# Autodesk Inventor assembly: 조립품2
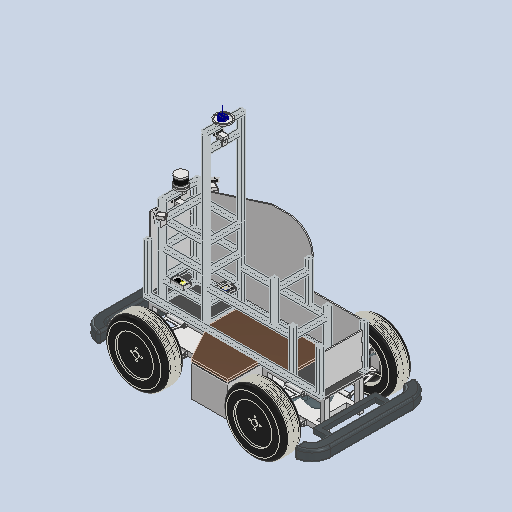
[picture p0: Inventor's stored thumbnail of the model, 512x512]
Saved by Autodesk Inventor 2025.2 (Build 292293000, 293)
## iProperties
Created: 2025-01-26
Part Number: 조립품2
Document SubType Name: Assembly
Designer: jbhma
Author: jbhma
## Documents named in this file (38)
- C:\Users\jbhma\OneDrive\Desktop\2025_ACCA\2024 ERP42\25_Car\Car - 복사본.iam
- C:\Users\jbhma\OneDrive\Desktop\2025_ACCA\2024 ERP42\body.ipt
- C:\Users\jbhma\OneDrive\Desktop\2025_ACCA\2024 ERP42\body_braket.ipt
- C:\Users\jbhma\OneDrive\Desktop\2025_ACCA\2024 ERP42\프로파일\40.5.ipt
- C:\Users\jbhma\OneDrive\Desktop\2025_ACCA\2024 ERP42\프로파일\71.ipt
- C:\Users\jbhma\OneDrive\Desktop\2025_ACCA\2024 ERP42\프로파일\34.ipt
- C:\Users\jbhma\OneDrive\Desktop\2025_ACCA\2024 ERP42\프로파일\26.ipt
- C:\Users\jbhma\OneDrive\Desktop\2025_ACCA\2024 ERP42\프로파일\79.ipt
- C:\Users\jbhma\OneDrive\Desktop\2025_ACCA\2024 ERP42\프로파일\39.ipt
- C:\Users\jbhma\OneDrive\Desktop\2025_ACCA\2024 ERP42\bumper.ipt
- C:\Users\jbhma\OneDrive\Desktop\2025_ACCA\2024 ERP42\link.ipt
- C:\Users\jbhma\OneDrive\Desktop\2025_ACCA\2024 ERP42\wheel_bolt.ipt
- C:\Users\jbhma\OneDrive\Desktop\2025_ACCA\2024 ERP42\wheel_braket_13.ipt
- C:\Users\jbhma\OneDrive\Desktop\2025_ACCA\2024 ERP42\wheel_braket_24.ipt
- C:\Users\jbhma\OneDrive\Desktop\2025_ACCA\2024 ERP42\wheel.ipt
- C:\Users\jbhma\OneDrive\Desktop\2025_ACCA\2024 ERP42\base_link.ipt
- base_link.ipt
- C:\Users\jbhma\OneDrive\Desktop\2025_ACCA\2024 ERP42\프로파일\50.ipt
- C:\Users\jbhma\OneDrive\Desktop\2025_ACCA\2024 ERP42\camera_case_front.ipt
- C:\Users\jbhma\OneDrive\Desktop\2025_ACCA\2024 ERP42\camera_case_left.ipt
- C:\Users\jbhma\OneDrive\Desktop\2025_ACCA\2024 ERP42\camera_case_right.ipt
- C:\Users\jbhma\OneDrive\Desktop\2025_ACCA\2024 ERP42\camera.ipt
- C:\Users\jbhma\OneDrive\Desktop\2025_ACCA\2024 ERP42\lidar_case.ipt
- C:\Users\jbhma\OneDrive\Desktop\2025_ACCA\2024 ERP42\imu_case_new.ipt
- C:\Users\jbhma\OneDrive\Desktop\2025_ACCA\2024 ERP42\gps_case.ipt
- C:\Users\jbhma\OneDrive\Desktop\2025_ACCA\2024 ERP42\UBLOX_ANN-MB-00_GNSS_ANTENNA.ipt
- C:\Users\jbhma\OneDrive\Desktop\2025_ACCA\2024 ERP42\lidar.ipt
- C:\Users\jbhma\OneDrive\Desktop\2025_ACCA\2024 ERP42\MTi 600-series STEP files\MTi-600 DEV assembly.iam
- C:\Users\jbhma\OneDrive\Desktop\2025_ACCA\2024 ERP42\MTi 600-series STEP files\MTi 1-s DK GNSS.iam
- C:\Users\jbhma\OneDrive\Desktop\2025_ACCA\2024 ERP42\gps_case_2.ipt
- C:\Users\jbhma\OneDrive\Desktop\2025_ACCA\2024 ERP42\gps_black.ipt
- C:\Users\jbhma\OneDrive\Desktop\2025_ACCA\2024 ERP42\cover.ipt
- C:\Users\jbhma\OneDrive\Desktop\2025_ACCA\2024 ERP42\고무커버.ipt
- C:\Users\jbhma\OneDrive\Desktop\2025_ACCA\2024 ERP42\프로파일\153.ipt
- C:\Users\jbhma\OneDrive\Desktop\2025_ACCA\2024 ERP42\side_cowl.ipt
- C:\Users\jbhma\OneDrive\Desktop\2025_ACCA\2024 ERP42\back_cowl.ipt
- C:\Users\jbhma\OneDrive\Desktop\2025_ACCA\2024 ERP42\fornt_cowl.ipt
- C:\Users\jbhma\OneDrive\Desktop\2025_ACCA\2024 ERP42\프로파일\34.5.ipt
## Components (101 placed, 36 different names)
1. body:1 — 메이트:113, 메이트:114, 메이트:115, 메이트:116, 메이트:117, 메이트:118, 메이트:119, 메이트:120, 메이트:124, 메이트:125, 메이트:126, 메이트:127, 메이트:128, 메이트:131, 메이트:137, 메이트:139, 메이트:159, 메이트:162, 메이트:191, 메이트:192, 메이트:193, 메이트:194, 메이트:195, 메이트:196, 메이트:197, 메이트:198, 메이트:199, 메이트:200, 메이트:201, 메이트:202, 메이트:203, 메이트:204, 메이트:205, 메이트:206, 메이트:303, 메이트:348, 메이트:349
2. body_braket:9 — 메이트:113, 메이트:114, 메이트:212
3. body_braket:10 — 메이트:115, 메이트:116, 메이트:211
4. body_braket:11 — 메이트:117, 메이트:118, 메이트:213
5. body_braket:12 — 메이트:119, 메이트:120, 메이트:214
6. body_braket:13 — 메이트:191, 메이트:195, 메이트:199, 메이트:215
7. body_braket:14 — 메이트:193, 메이트:197, 메이트:202, 메이트:217
8. body_braket:15 — 메이트:194, 메이트:198, 메이트:201, 메이트:218
9. body_braket:16 — 메이트:192, 메이트:196, 메이트:200, 메이트:216
10. bumper:1 — 메이트:203, 메이트:204
11. bumper:2 — 메이트:205, 메이트:206
12. 40.5:12 — 메이트:126, 메이트:127, 메이트:130, 메이트:257
13. 40.5:13 — 메이트:124, 메이트:125, 메이트:129
14. 71:1 — 메이트:128, 메이트:129, 메이트:132, 메이트:133, 메이트:138
15. 71:2 — 메이트:130, 메이트:131, 메이트:134, 메이트:135, 메이트:136, 메이트:256
16. 34:1 — 메이트:134, 메이트:135, 메이트:189
17. 34:2 — 메이트:132, 메이트:133, 메이트:190
18. 40.5:15 — 메이트:136, 메이트:137, 메이트:143, 메이트:144, 메이트:145, 메이트:326
19. 40.5:16 — 메이트:138, 메이트:139, 메이트:140, 메이트:141, 메이트:142, 메이트:155, 메이트:287, 메이트:288, 메이트:324, 메이트:332
20. 26:1 — 메이트:140, 메이트:141, 메이트:142, 메이트:149, 메이트:150, 메이트:156, 메이트:175, 메이트:176, 메이트:178
21. 26:2 — 메이트:143, 메이트:144, 메이트:145, 메이트:151, 메이트:152, 메이트:157, 메이트:158, 메이트:177
22. 79:1 — 메이트:151, 메이트:152, 메이트:261
23. 79:2 — 메이트:149, 메이트:150, 메이트:153, 메이트:154, 메이트:262, 각도:3
24. 34:3 — 메이트:153, 메이트:154, 메이트:259
25. 34:4 — 메이트:155, 메이트:156, 메이트:160, 메이트:174
26. 34:5 — 메이트:157, 메이트:158, 메이트:161
27. 40.5:17 — 메이트:161, 메이트:162, 메이트:163, 메이트:164, 메이트:282, 메이트:304
28. 40.5:18 — 메이트:159, 메이트:160, 메이트:165, 메이트:166, 메이트:283, 메이트:330
29. 39:1 — 메이트:163, 메이트:164, 메이트:183, 메이트:187
30. 39:2 — 메이트:165, 메이트:166, 메이트:173, 메이트:185, 메이트:252, 메이트:253, 메이트:266, 메이트:347
31. 26:4 — 메이트:173, 메이트:174
32. 26:5 — 메이트:175, 메이트:176
33. 26:6 — 메이트:177, 메이트:178, 메이트:182, 메이트:184
34. 26:8 — 메이트:258, 메이트:261, 메이트:262
35. 34:8 — 메이트:182, 메이트:183
36. 34:9 — 메이트:184, 메이트:185, 메이트:186, 메이트:240, 플러쉬:1
37. 26:9 — 메이트:186, 메이트:187, 메이트:239
38. 26:10 — 메이트:189, 메이트:190
39. link:5 — 메이트:211, 메이트:226
40. link:6 — 메이트:212, 메이트:224
41. link:7 — 메이트:214, 메이트:227
42. link:8 — 메이트:213, 메이트:225
43. link:12 — 메이트:215, 메이트:219
44. link:13 — 메이트:217, 메이트:223
45. link:14 — 메이트:216, 메이트:220
46. link:15 — 메이트:218, 메이트:222
47. wheel_bolt:1 — 메이트:219, 메이트:221
48. wheel_braket_13:1 — 메이트:221, 메이트:236, 메이트:237
49. wheel_braket_24:1 — 메이트:229, 메이트:235, 메이트:238
50. wheel_bolt:2 — 메이트:220
51. wheel_bolt:3 — 메이트:222, 메이트:230
52. wheel_bolt:4 — 메이트:223
53. wheel_bolt:5 — 메이트:224, 메이트:228
54. wheel_bolt:6 — 메이트:225, 메이트:229
55. wheel_bolt:7 — 메이트:226
56. wheel_bolt:8 — 메이트:227
57. wheel_braket_13:2 — 메이트:228, 메이트:232
58. wheel:1 — 메이트:232
59. wheel:2 — 메이트:238
60. wheel_braket_24:2 — 메이트:230, 메이트:234
61. wheel:3 — 메이트:237
62. wheel:4 — 메이트:234
63. base_link:1 — 메이트:235, 메이트:236
64. 50:1 — 메이트:240, 플러쉬:1, 메이트:241, 메이트:242, 메이트:243, 메이트:244, 메이트:245
65. camera_case_front:1 — 메이트:239, 메이트:241, 메이트:246, 메이트:247, 메이트:266
66. camera_case_left:1 — 메이트:242, 메이트:243, 메이트:250, 메이트:251
67. camera_case_right:1 — 메이트:244, 메이트:245, 메이트:248, 메이트:249
68. camera:1 — 메이트:246, 메이트:247
69. camera:2 — 메이트:248, 메이트:249
70. camera:3 — 메이트:250, 메이트:251
71. 26:11 — 메이트:252, 메이트:253, 메이트:346
72. 26:12 — 메이트:256, 메이트:257
73. gps_case:1 — 메이트:259, 각도:3
74. camera_case_front:2 — 메이트:258, 메이트:278
75. UBLOX_ANN-MB-00_GNSS_ANTENNA:1
76. camera:4 — 메이트:278
77. 26:13 — 메이트:282, 메이트:283
78. 26:14 — 메이트:287, 메이트:288
79. 34:10 — 메이트:303, 메이트:304
80. 34:15 — 메이트:324, 메이트:328
81. 34:16 — 메이트:326
82. gps_case_2:1 — 메이트:328, 메이트:338, 메이트:339
83. 26:17 — 메이트:330
84. MTi-600 DEV assembly:1 [sub-assembly] — 메이트:335, 메이트:336
85. imu_case_new:1 — 메이트:334, 메이트:335, 메이트:336
86. 26:18 — 메이트:332, 메이트:334
87. MTi 1-s DK GNSS:1 [sub-assembly] — 메이트:340
88. gps_black:1 — 메이트:338, 메이트:339, 메이트:340
89. lidar:3 — 회전:1
90. lidar_case:2 — 메이트:346, 메이트:347, 회전:1
91. cover:1 — 메이트:350, 메이트:351
92. 고무커버:1 — 메이트:348, 메이트:349, 메이트:350, 메이트:351, 메이트:352, 메이트:353, 메이트:354, 메이트:355
93. 153:1 — 메이트:354, 메이트:355, 메이트:361, 메이트:362, 메이트:375, 메이트:379, 메이트:384, 메이트:385, 메이트:386
94. 153:2 — 메이트:352, 메이트:353, 메이트:360, 메이트:363, 메이트:373, 메이트:380, 메이트:381, 메이트:382, 메이트:383
95. 40.5:21 — 메이트:360, 메이트:363, 메이트:374
96. 40.5:22 — 메이트:361, 메이트:362
97. back_cowl:1 — 메이트:373
98. fornt_cowl:1 — 메이트:374, 메이트:375
99. side_cowl:1 — 메이트:379
100. 34.5:1 — 메이트:380, 메이트:381, 메이트:382, 메이트:383
101. 34.5:2 — 메이트:384, 메이트:385, 메이트:386
## Relationships (172: Mate 169, Flush 1, Angle 1, RevoluteJoint 1)
- 메이트:113 [Mate] (195 mm): body:1 ↔ body_braket:9
- 메이트:114 [Mate]: body:1 ↔ body_braket:9
- 메이트:115 [Mate] (195 mm): body:1 ↔ body_braket:10
- 메이트:116 [Mate]: body:1 ↔ body_braket:10
- 메이트:117 [Mate] (155 mm): body:1 ↔ body_braket:11
- 메이트:118 [Mate]: body:1 ↔ body_braket:11
- 메이트:119 [Mate] (155 mm): body:1 ↔ body_braket:12
- 메이트:120 [Mate]: body:1 ↔ body_braket:12
- 메이트:124 [Mate]: body:1 ↔ 40.5:13
- 메이트:125 [Mate] (275 mm): body:1 ↔ 40.5:13
- 메이트:126 [Mate]: body:1 ↔ 40.5:12
- 메이트:127 [Mate] (275 mm): body:1 ↔ 40.5:12
- 메이트:128 [Mate] (300 mm): body:1 ↔ 71:1
- 메이트:129 [Mate]: 40.5:13 ↔ 71:1
- 메이트:130 [Mate]: 40.5:12 ↔ 71:2
- 메이트:131 [Mate] (300 mm): body:1 ↔ 71:2
- 메이트:132 [Mate]: 71:1 ↔ 34:2
- 메이트:133 [Mate] (120 mm): 71:1 ↔ 34:2
- 메이트:134 [Mate]: 71:2 ↔ 34:1
- 메이트:135 [Mate] (120 mm): 71:2 ↔ 34:1
- 메이트:136 [Mate]: 71:2 ↔ 40.5:15
- 메이트:137 [Mate]: body:1 ↔ 40.5:15
- 메이트:138 [Mate]: 71:1 ↔ 40.5:16
- 메이트:139 [Mate]: body:1 ↔ 40.5:16
- 메이트:140 [Mate]: 40.5:16 ↔ 26:1
- 메이트:141 [Mate]: 40.5:16 ↔ 26:1
- 메이트:142 [Mate]: 40.5:16 ↔ 26:1
- 메이트:143 [Mate]: 40.5:15 ↔ 26:2
- 메이트:144 [Mate]: 40.5:15 ↔ 26:2
- 메이트:145 [Mate]: 40.5:15 ↔ 26:2
- 메이트:149 [Mate]: 26:1 ↔ 79:2
- 메이트:150 [Mate]: 26:1 ↔ 79:2
- 메이트:151 [Mate]: 26:2 ↔ 79:1
- 메이트:152 [Mate]: 26:2 ↔ 79:1
- 메이트:153 [Mate]: 79:2 ↔ 34:3
- 메이트:154 [Mate]: 79:2 ↔ 34:3
- 메이트:155 [Mate]: 40.5:16 ↔ 34:4
- 메이트:156 [Mate]: 26:1 ↔ 34:4
- 메이트:157 [Mate]: 26:2 ↔ 34:5
- 메이트:158 [Mate]: 26:2 ↔ 34:5
- 메이트:159 [Mate]: body:1 ↔ 40.5:18
- 메이트:160 [Mate]: 34:4 ↔ 40.5:18
- 메이트:161 [Mate]: 34:5 ↔ 40.5:17
- 메이트:162 [Mate]: body:1 ↔ 40.5:17
- 메이트:163 [Mate]: 40.5:17 ↔ 39:1
- 메이트:164 [Mate]: 40.5:17 ↔ 39:1
- 메이트:165 [Mate]: 40.5:18 ↔ 39:2
- 메이트:166 [Mate]: 40.5:18 ↔ 39:2
- 메이트:173 [Mate]: 39:2 ↔ 26:4
- 메이트:174 [Mate]: 34:4 ↔ 26:4
- 메이트:175 [Mate]: 26:1 ↔ 26:5
- 메이트:176 [Mate]: 26:1 ↔ 26:5
- 메이트:177 [Mate]: 26:2 ↔ 26:6
- 메이트:178 [Mate]: 26:1 ↔ 26:6
- 메이트:182 [Mate]: 26:6 ↔ 34:8
- 메이트:183 [Mate]: 39:1 ↔ 34:8
- 메이트:184 [Mate]: 26:6 ↔ 34:9
- 메이트:185 [Mate]: 39:2 ↔ 34:9
- 메이트:186 [Mate]: 34:9 ↔ 26:9
- 메이트:187 [Mate]: 39:1 ↔ 26:9
- 메이트:189 [Mate]: 34:1 ↔ 26:10
- 메이트:190 [Mate]: 34:2 ↔ 26:10
- 메이트:191 [Mate]: body:1 ↔ body_braket:13
- 메이트:192 [Mate]: body:1 ↔ body_braket:16
- 메이트:193 [Mate]: body:1 ↔ body_braket:14
- 메이트:194 [Mate]: body:1 ↔ body_braket:15
- 메이트:195 [Mate]: body:1 ↔ body_braket:13
- 메이트:196 [Mate]: body:1 ↔ body_braket:16
- 메이트:197 [Mate]: body:1 ↔ body_braket:14
- 메이트:198 [Mate]: body:1 ↔ body_braket:15
- 메이트:199 [Mate] (155 mm): body:1 ↔ body_braket:13
- 메이트:200 [Mate] (155 mm): body:1 ↔ body_braket:16
- 메이트:201 [Mate] (195 mm): body:1 ↔ body_braket:15
- 메이트:202 [Mate] (195 mm): body:1 ↔ body_braket:14
- 메이트:203 [Mate]: body:1 ↔ bumper:1
- 메이트:204 [Mate] (100 mm): body:1 ↔ bumper:1
- 메이트:205 [Mate]: body:1 ↔ bumper:2
- 메이트:206 [Mate] (100 mm): body:1 ↔ bumper:2
- 메이트:211 [Mate]: body_braket:10 ↔ link:5
- 메이트:212 [Mate]: body_braket:9 ↔ link:6
- 메이트:213 [Mate]: body_braket:11 ↔ link:8
- 메이트:214 [Mate]: body_braket:12 ↔ link:7
- 메이트:215 [Mate]: body_braket:13 ↔ link:12
- 메이트:216 [Mate]: body_braket:16 ↔ link:14
- 메이트:217 [Mate]: body_braket:14 ↔ link:13
- 메이트:218 [Mate]: body_braket:15 ↔ link:15
- 메이트:219 [Mate]: link:12 ↔ wheel_bolt:1
- 메이트:220 [Mate]: link:14 ↔ wheel_bolt:2
- 메이트:221 [Mate]: wheel_bolt:1 ↔ wheel_braket_13:1
- 메이트:222 [Mate]: link:15 ↔ wheel_bolt:3
- 메이트:223 [Mate]: link:13 ↔ wheel_bolt:4
- 메이트:224 [Mate]: link:6 ↔ wheel_bolt:5
- 메이트:225 [Mate]: link:8 ↔ wheel_bolt:6
- 메이트:226 [Mate]: link:5 ↔ wheel_bolt:7
- 메이트:227 [Mate]: link:7 ↔ wheel_bolt:8
- 메이트:228 [Mate]: wheel_bolt:5 ↔ wheel_braket_13:2
- 메이트:229 [Mate]: wheel_braket_24:1 ↔ wheel_bolt:6
- 메이트:230 [Mate]: wheel_bolt:3 ↔ wheel_braket_24:2
- 메이트:232 [Mate]: wheel_braket_13:2 ↔ wheel:1
- 메이트:234 [Mate]: wheel_braket_24:2 ↔ wheel:4
- 메이트:235 [Mate]: wheel_braket_24:1 ↔ base_link:1
- 메이트:236 [Mate]: wheel_braket_13:1 ↔ base_link:1
- 메이트:237 [Mate]: wheel_braket_13:1 ↔ wheel:3
- 메이트:238 [Mate]: wheel_braket_24:1 ↔ wheel:2
- 메이트:239 [Mate]: 26:9 ↔ camera_case_front:1
- 메이트:240 [Mate]: 34:9 ↔ 50:1
- 플러쉬:1 [Flush] (-80 mm): 34:9 ↔ 50:1
- 메이트:241 [Mate]: 50:1 ↔ camera_case_front:1
- 메이트:242 [Mate]: 50:1 ↔ camera_case_left:1
- 메이트:243 [Mate]: 50:1 ↔ camera_case_left:1
- 메이트:244 [Mate]: 50:1 ↔ camera_case_right:1
- 메이트:245 [Mate]: 50:1 ↔ camera_case_right:1
- 메이트:246 [Mate]: camera_case_front:1 ↔ camera:1
- 메이트:247 [Mate]: camera_case_front:1 ↔ camera:1
- 메이트:248 [Mate]: camera_case_right:1 ↔ camera:2
- 메이트:249 [Mate]: camera_case_right:1 ↔ camera:2
- 메이트:250 [Mate]: camera_case_left:1 ↔ camera:3
- 메이트:251 [Mate]: camera_case_left:1 ↔ camera:3
- 메이트:252 [Mate]: 39:2 ↔ 26:11
- 메이트:253 [Mate]: 39:2 ↔ 26:11
- 메이트:256 [Mate]: 71:2 ↔ 26:12
- 메이트:257 [Mate]: 40.5:12 ↔ 26:12
- 메이트:258 [Mate]: 26:8 ↔ camera_case_front:2
- 메이트:259 [Mate]: 34:3 ↔ gps_case:1
- 메이트:261 [Mate]: 79:1 ↔ 26:8
- 메이트:262 [Mate]: 79:2 ↔ 26:8
- 각도:3 [Angle] (90 deg): 79:2 ↔ gps_case:1
- 메이트:266 [Mate] (106 mm): 39:2 ↔ camera_case_front:1
- 메이트:278 [Mate]: camera_case_front:2 ↔ camera:4
- 메이트:282 [Mate]: 40.5:17 ↔ 26:13
- 메이트:283 [Mate]: 40.5:18 ↔ 26:13
- 메이트:287 [Mate]: 40.5:16 ↔ 26:14
- 메이트:288 [Mate]: 40.5:16 ↔ 26:14
- 메이트:303 [Mate]: body:1 ↔ 34:10
- 메이트:304 [Mate]: 40.5:17 ↔ 34:10
- 메이트:324 [Mate]: 40.5:16 ↔ 34:15
- 메이트:326 [Mate]: 40.5:15 ↔ 34:16
- 메이트:328 [Mate]: 34:15 ↔ gps_case_2:1
- 메이트:330 [Mate]: 40.5:18 ↔ 26:17
- 메이트:332 [Mate]: 40.5:16 ↔ 26:18
- 메이트:334 [Mate]: imu_case_new:1 ↔ 26:18
- 메이트:335 [Mate]: MTi-600 DEV assembly:1 ↔ imu_case_new:1
- 메이트:336 [Mate]: MTi-600 DEV assembly:1 ↔ imu_case_new:1
- 메이트:338 [Mate]: gps_case_2:1 ↔ gps_black:1
- 메이트:339 [Mate]: gps_case_2:1 ↔ gps_black:1
- 메이트:340 [Mate]: MTi 1-s DK GNSS:1 ↔ gps_black:1
- 메이트:346 [Mate]: 26:11 ↔ lidar_case:2
- 메이트:347 [Mate] (120 mm): 39:2 ↔ lidar_case:2
- 회전:1 [RevoluteJoint]: lidar:3 ↔ lidar_case:2
- 메이트:348 [Mate]: body:1 ↔ 고무커버:1
- 메이트:349 [Mate]: body:1 ↔ 고무커버:1
- 메이트:350 [Mate]: cover:1 ↔ 고무커버:1
- 메이트:351 [Mate]: cover:1 ↔ 고무커버:1
- 메이트:352 [Mate]: 고무커버:1 ↔ 153:2
- 메이트:353 [Mate]: 고무커버:1 ↔ 153:2
- 메이트:354 [Mate]: 고무커버:1 ↔ 153:1
- 메이트:355 [Mate]: 고무커버:1 ↔ 153:1
- 메이트:360 [Mate]: 153:2 ↔ 40.5:21
- 메이트:361 [Mate]: 153:1 ↔ 40.5:22
- 메이트:362 [Mate]: 153:1 ↔ 40.5:22
- 메이트:363 [Mate]: 153:2 ↔ 40.5:21
- 메이트:373 [Mate]: 153:2 ↔ back_cowl:1
- 메이트:374 [Mate]: 40.5:21 ↔ fornt_cowl:1
- 메이트:375 [Mate]: 153:1 ↔ fornt_cowl:1
- 메이트:379 [Mate]: 153:1 ↔ side_cowl:1
- 메이트:380 [Mate]: 153:2 ↔ 34.5:1
- 메이트:381 [Mate]: 153:2 ↔ 34.5:1
- 메이트:382 [Mate]: 153:2 ↔ 34.5:1
- 메이트:383 [Mate]: 153:2 ↔ 34.5:1
- 메이트:384 [Mate]: 153:1 ↔ 34.5:2
- 메이트:385 [Mate]: 153:1 ↔ 34.5:2
- 메이트:386 [Mate]: 153:1 ↔ 34.5:2
